# Autodesk Inventor assembly: ENSAMBLAJE_VENTOSA_2
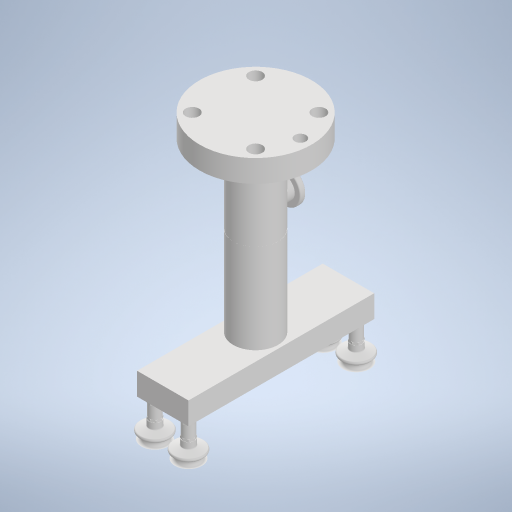
[picture p0: Inventor's stored thumbnail of the model, 512x512]
Saved by Autodesk Inventor 2024 (Build 280153000, 153)
## iProperties
Created: 2022-10-31
Part Number: ENSAMBLAJE_VENTOSA_2
Document SubType Name: Assembly
Designer: Usuario
Mass: 57.9805 g
Surface Area: 254.277 cm^2
Volume: 57.9805 cm^3
Author: Usuario
## Documents named in this file (15)
- C:\Users\sebas\OneDrive\Documentos\Cosas de Sebastian\APM\Esdek\Celda Robotizada\ROBOT STUDIO\CAD\HERRAMIENTA\ENSAMBLAJE_VENTOSA_2.iam
- C:\Users\sebas\OneDrive\Documentos\Cosas de Sebastian\APM\Esdek\Celda Robotizada\ROBOT STUDIO\CAD\HERRAMIENTA\ACOPLE.ipt
- C:\Users\sebas\OneDrive\Documentos\Cosas de Sebastian\APM\Esdek\Celda Robotizada\ROBOT STUDIO\CAD\HERRAMIENTA\TORNILLO_B.ipt
- C:\Users\sebas\OneDrive\Documentos\Cosas de Sebastian\APM\Esdek\Celda Robotizada\ROBOT STUDIO\CAD\HERRAMIENTA\TUBO_METALICO_B.ipt
- C:\Users\sebas\OneDrive\Documentos\Cosas de Sebastian\APM\Esdek\Celda Robotizada\ROBOT STUDIO\CAD\HERRAMIENTA\VENTOSA_B.ipt
- C:\Users\sebas\OneDrive\Documentos\Cosas de Sebastian\APM\Esdek\Celda Robotizada\ROBOT STUDIO\CAD\HERRAMIENTA\UNION_B.ipt
- C:\Users\sebas\OneDrive\Documentos\Cosas de Sebastian\APM\Esdek\Celda Robotizada\ROBOT STUDIO\CAD\HERRAMIENTA\TORNILLO_B_MIR.ipt
- C:\Users\sebas\OneDrive\Documentos\Cosas de Sebastian\APM\Esdek\Celda Robotizada\ROBOT STUDIO\CAD\HERRAMIENTA\TUBO_METALICO_B_MIR.ipt
- C:\Users\sebas\OneDrive\Documentos\Cosas de Sebastian\APM\Esdek\Celda Robotizada\ROBOT STUDIO\CAD\HERRAMIENTA\VENTOSA_B_MIR.ipt
- C:\Users\sebas\OneDrive\Documentos\Cosas de Sebastian\APM\Esdek\Celda Robotizada\ROBOT STUDIO\CAD\HERRAMIENTA\TORNILLO_B_MIR1.ipt
- C:\Users\sebas\OneDrive\Documentos\Cosas de Sebastian\APM\Esdek\Celda Robotizada\ROBOT STUDIO\CAD\HERRAMIENTA\TUBO_METALICO_B_MIR1.ipt
- C:\Users\sebas\OneDrive\Documentos\Cosas de Sebastian\APM\Esdek\Celda Robotizada\ROBOT STUDIO\CAD\HERRAMIENTA\VENTOSA_B_MIR1.ipt
- C:\Users\sebas\OneDrive\Documentos\Cosas de Sebastian\APM\Esdek\Celda Robotizada\ROBOT STUDIO\CAD\HERRAMIENTA\TORNILLO_B_MIR_MIR.ipt
- C:\Users\sebas\OneDrive\Documentos\Cosas de Sebastian\APM\Esdek\Celda Robotizada\ROBOT STUDIO\CAD\HERRAMIENTA\TUBO_METALICO_B_MIR_MIR.ipt
- C:\Users\sebas\OneDrive\Documentos\Cosas de Sebastian\APM\Esdek\Celda Robotizada\ROBOT STUDIO\CAD\HERRAMIENTA\VENTOSA_B_MIR_MIR.ipt
## Components (14 placed, 14 different names)
1. ACOPLE:1 — Coincidencia:9, Coincidencia:10, Coincidencia:11, De rotación:7, Coincidencia:16
2. TORNILLO_B:4 — Cilíndrica:1, De rotación:15, De rotación:16
3. TUBO_METALICO_B:4 — Cilíndrica:1, Coincidencia:15
4. VENTOSA_B:4 — De rotación:16
5. UNION_B:1 — De rotación:7, De rotación:10, De rotación:11, Coincidencia:12, Coincidencia:13, De rotación:13, Coincidencia:14, De rotación:15, Coincidencia:15, Coincidencia:17
6. TORNILLO_B_MIR:1 — Cilíndrica:2, De rotación:13, De rotación:14
7. TUBO_METALICO_B_MIR:1 — Cilíndrica:2, Coincidencia:14
8. VENTOSA_B_MIR:1 — De rotación:14
9. TORNILLO_B_MIR1:1 — Cilíndrica:3, De rotación:11, De rotación:12
10. TUBO_METALICO_B_MIR1:1 — Cilíndrica:3, Coincidencia:12
11. VENTOSA_B_MIR1:1 — De rotación:12
12. TORNILLO_B_MIR_MIR:1 — De rotación:8, De rotación:10, Cilíndrica:4
13. TUBO_METALICO_B_MIR_MIR:1 — Cilíndrica:4, Coincidencia:13
14. VENTOSA_B_MIR_MIR:1 — De rotación:8
## Relationships (22: Mate 9, RevoluteJoint 9, CylindricalJoint 4)
- Cilíndrica:1 [CylindricalJoint]: TORNILLO_B:4 ↔ TUBO_METALICO_B:4
- Cilíndrica:2 [CylindricalJoint]: TORNILLO_B_MIR:1 ↔ TUBO_METALICO_B_MIR:1
- Cilíndrica:3 [CylindricalJoint]: TORNILLO_B_MIR1:1 ↔ TUBO_METALICO_B_MIR1:1
- Coincidencia:9 [Mate]: ACOPLE:1
- Coincidencia:10 [Mate]: ACOPLE:1
- Coincidencia:11 [Mate]: ACOPLE:1
- De rotación:7 [RevoluteJoint]: ACOPLE:1 ↔ UNION_B:1
- De rotación:8 [RevoluteJoint] (-1 mm): TORNILLO_B_MIR_MIR:1 ↔ VENTOSA_B_MIR_MIR:1
- De rotación:10 [RevoluteJoint] (-4 mm): UNION_B:1 ↔ TORNILLO_B_MIR_MIR:1
- De rotación:11 [RevoluteJoint] (4 mm): UNION_B:1 ↔ TORNILLO_B_MIR1:1
- De rotación:12 [RevoluteJoint] (1 mm): TORNILLO_B_MIR1:1 ↔ VENTOSA_B_MIR1:1
- Coincidencia:12 [Mate]: UNION_B:1 ↔ TUBO_METALICO_B_MIR1:1
- Cilíndrica:4 [CylindricalJoint]: TORNILLO_B_MIR_MIR:1 ↔ TUBO_METALICO_B_MIR_MIR:1
- Coincidencia:13 [Mate]: UNION_B:1 ↔ TUBO_METALICO_B_MIR_MIR:1
- De rotación:13 [RevoluteJoint] (4 mm): UNION_B:1 ↔ TORNILLO_B_MIR:1
- Coincidencia:14 [Mate]: UNION_B:1 ↔ TUBO_METALICO_B_MIR:1
- De rotación:14 [RevoluteJoint] (1 mm): TORNILLO_B_MIR:1 ↔ VENTOSA_B_MIR:1
- De rotación:15 [RevoluteJoint] (4 mm): TORNILLO_B:4 ↔ UNION_B:1
- De rotación:16 [RevoluteJoint] (-1 mm): TORNILLO_B:4 ↔ VENTOSA_B:4
- Coincidencia:15 [Mate]: TUBO_METALICO_B:4 ↔ UNION_B:1
- Coincidencia:16 [Mate]: ACOPLE:1
- Coincidencia:17 [Mate] (-11.5 mm): UNION_B:1
